# Autodesk Inventor assembly: microservoAssembly
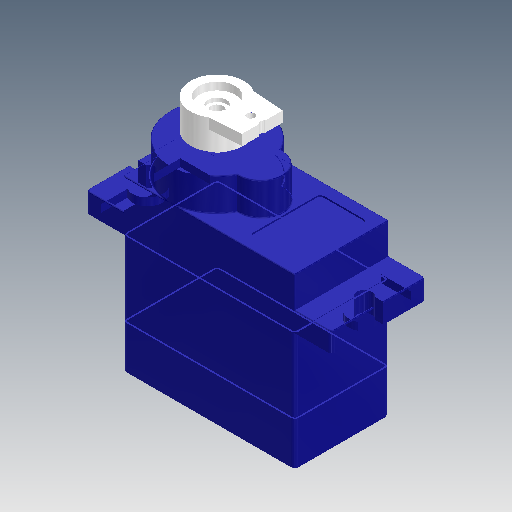
[picture p0: Inventor's stored thumbnail of the model, 512x512]
Saved by Autodesk Inventor 2020.3 (Build 243373000, 373)
## iProperties
Created: 2019-10-22
Part Number: microservoAssembly
Document SubType Name: Assembly
Designer: justi
Mass: 9.10844 g
Surface Area: 30.4057 cm^2
Volume: 7.19704 cm^3
Density: 1.26558 g/cm^3
Sending System: SolidWorks 2018
Last Author: DuctopwH
Last Saved: 2019-10-25
Author: justi
## Documents named in this file (3)
- F:\UQ Engineering\2021 ~ 5th Year\Semester 2\METR4911-THESIS\FarmBot CAD\FarmBotV1\tower-pro-sg90-micro-servo\microservoAssembly.iam
- F:\UQ Engineering\2021 ~ 5th Year\Semester 2\METR4911-THESIS\FarmBot CAD\FarmBotV1\tower-pro-sg90-micro-servo\microservoSG90.ipt
- F:\UQ Engineering\2021 ~ 5th Year\Semester 2\METR4911-THESIS\FarmBot CAD\FarmBotV1\tower-pro-sg90-micro-servo\microservoArm.ipt
## Components (2 placed, 2 different names)
1. microservoSG90:1 — Mate:1, Mate:2, Mate:3
2. microservoArm:1 — Mate:1, Mate:2, Mate:3
## Relationships (3: Mate 3)
- Mate:1: microservoSG90:1 ↔ microservoArm:1
- Mate:2: microservoSG90:1 ↔ microservoArm:1
- Mate:3: microservoSG90:1 ↔ microservoArm:1
